# Autodesk Inventor assembly: Корпус ноги в сборе
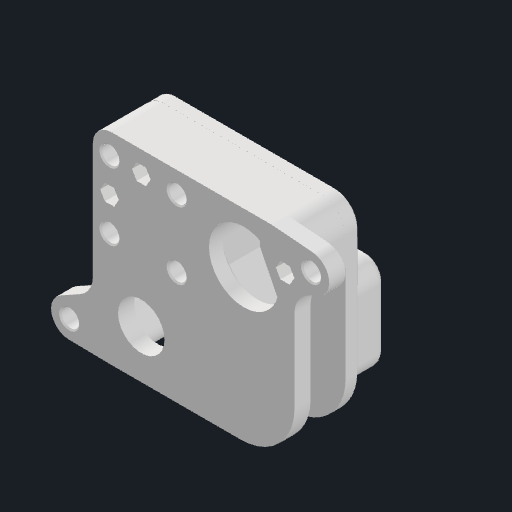
[picture p0: Inventor's stored thumbnail of the model, 512x512]
Saved by Autodesk Inventor 2025 (Build 290162010, 162A)
## iProperties
Created: 2025-01-17
Part Number: Корпус ноги в сборе
Document SubType Name: Assembly
Designer: Edward_Higgins
Author: Edward_Higgins
## Documents named in this file (4)
- D:\Users\Edward_Higgins\Desktop\ZAVOD\TWR2\Корпус ноги в сборе.iam
- D:\Users\Edward_Higgins\Desktop\ZAVOD\TWR2\Корпус ноги 2.ipt
- D:\Users\Edward_Higgins\Desktop\ZAVOD\TWR2\Пластина корпуса ноги.ipt
- D:\Users\Edward_Higgins\Desktop\ZAVOD\TWR2\Стандартные детали\Винт М3х19.ipt
## Components (5 placed, 3 different names)
1. Корпус ноги 2:1 — Совмещение:1, Совмещение:2, Совмещение:3, Совмещение:4, Совмещение:5, Совмещение:6, Совмещение:7, Совмещение:9, Совмещение:10, Совмещение:11, Совмещение:12
2. Пластина корпуса ноги:1 — Совмещение:3, Совмещение:4, Совмещение:5
3. Винт М3х19:2 — Совмещение:6, Совмещение:7
4. Винт М3х19:3 — Совмещение:11, Совмещение:12
5. Винт М3х19:4 — Совмещение:9, Совмещение:10
## Relationships (11: Mate 11)
- Совмещение:1 [Mate]: Корпус ноги 2:1
- Совмещение:2 [Mate]: Корпус ноги 2:1
- Совмещение:3 [Mate]: Корпус ноги 2:1 ↔ Пластина корпуса ноги:1
- Совмещение:4 [Mate]: Корпус ноги 2:1 ↔ Пластина корпуса ноги:1
- Совмещение:5 [Mate]: Корпус ноги 2:1 ↔ Пластина корпуса ноги:1
- Совмещение:6 [Mate]: Корпус ноги 2:1 ↔ Винт М3х19:2
- Совмещение:7 [Mate]: Корпус ноги 2:1 ↔ Винт М3х19:2
- Совмещение:9 [Mate]: Корпус ноги 2:1 ↔ Винт М3х19:4
- Совмещение:10 [Mate]: Корпус ноги 2:1 ↔ Винт М3х19:4
- Совмещение:11 [Mate]: Корпус ноги 2:1 ↔ Винт М3х19:3
- Совмещение:12 [Mate]: Корпус ноги 2:1 ↔ Винт М3х19:3
